# Autodesk Inventor assembly: 0002_Tam_nguyen_Truc_Z
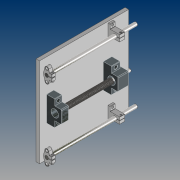
[picture p0: Inventor's stored thumbnail of the model, 180x180]
Saved by Autodesk Inventor 2021 (Build 250183000, 183)
## iProperties
Created: 2024-04-08
Part Number: 0002_Tam_nguyen_Truc_Z
Document SubType Name: Assembly
Designer: Admin
Author: Admin
## Documents named in this file (6)
- C:\Users\Admin\Desktop\DO_AN_TOT_NGHIEP_2024\Mechanical\Design_in_3D\Version_2\0002_Tam_nguyen_Truc_Z.iam
- C:\Users\Admin\Desktop\DO_AN_TOT_NGHIEP_2024\Mechanical\Design_in_3D\Version_2\0002_Truc_Z.iam
- C:\Users\Admin\Desktop\DO_AN_TOT_NGHIEP_2024\Mechanical\Design_in_3D\Version_2\08_Tam_truc_Z.ipt
- C:\Users\Admin\Desktop\DO_AN_TOT_NGHIEP_2024\Mechanical\Design_in_3D\Library\sk10-3.snapshot.2\SK10.ipt
- C:\Users\Admin\Desktop\DO_AN_TOT_NGHIEP_2024\Mechanical\Design_in_3D\Version_2\09_Truc_song_song_x10x250.ipt
- C:\Users\Admin\Desktop\DO_AN_TOT_NGHIEP_2024\Mechanical\Design_in_3D\Library\shf10-shf8-linear-shaft-support-1.snapshot.6\SHF8.ipt
## Components (8 placed, 5 different names)
1. 0002_Truc_Z:1 [sub-assembly] — Mate:1, Mate:2, Angle:1, Mate:5
2. 08_Tam_truc_Z:1 — Mate:1, Mate:2, Mate:3, Mate:4, Angle:2, Flush:6
3. SK10:1 — Mate:3, Flush:1, Mate:5, Symmetry:1, Mate:6
4. SK10:2 — Mate:4, Angle:1, Flush:1, Symmetry:1, Mate:7
5. 09_Truc_song_song_x10x250:1 — Mate:7, Flush:2, Mate:8, Flush:5
6. 09_Truc_song_song_x10x250:2 — Mate:6, Flush:2, Mate:9
7. SHF8:1 — Flush:3, Mate:8, Angle:2, Flush:4, Flush:5, Flush:6
8. SHF8:2 — Flush:3, Mate:9, Flush:4
## Relationships (18: Mate 9, Flush 6, Angle 2, Symmetry 1)
- Mate:1: 0002_Truc_Z:1 ↔ 08_Tam_truc_Z:1
- Mate:2: 0002_Truc_Z:1 ↔ 08_Tam_truc_Z:1
- Mate:3: 08_Tam_truc_Z:1 ↔ SK10:1
- Mate:4: 08_Tam_truc_Z:1 ↔ SK10:2
- Angle:1 (0 deg): 0002_Truc_Z:1 ↔ SK10:2
- Flush:1: SK10:1 ↔ SK10:2
- Mate:5 (100 mm): 0002_Truc_Z:1 ↔ SK10:1
- Symmetry:1: SK10:1 ↔ SK10:2
- Mate:6: SK10:1 ↔ 09_Truc_song_song_x10x250:2
- Mate:7: SK10:2 ↔ 09_Truc_song_song_x10x250:1
- Flush:2: 09_Truc_song_song_x10x250:1 ↔ 09_Truc_song_song_x10x250:2
- Flush:3: SHF8:1 ↔ SHF8:2
- Mate:8: 09_Truc_song_song_x10x250:1 ↔ SHF8:1
- Angle:2 (0 deg): 08_Tam_truc_Z:1 ↔ SHF8:1
- Mate:9: 09_Truc_song_song_x10x250:2 ↔ SHF8:2
- Flush:4: SHF8:1 ↔ SHF8:2
- Flush:5: 09_Truc_song_song_x10x250:1 ↔ SHF8:1
- Flush:6: 08_Tam_truc_Z:1 ↔ SHF8:1
